# Autodesk Inventor assembly: CyberOrto
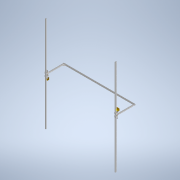
[picture p0: Inventor's stored thumbnail of the model, 180x180]
Saved by Autodesk Inventor 2022 (Build 260153000, 153)
## iProperties
RuleStatus: InUse
Created: 2021-12-29
Part Number: CyberOrto
Document SubType Name: Assembly
Designer: matte
Author: matte
## Documents named in this file (23)
- C:\Users\Elia\Documents\ELIA\UNITN\MAGISTRALE\1st year\1st semester\Mechanical Design\MDM-CyberOrto-CAD\CyberOrto.iam
- C:\Users\Elia\Documents\ELIA\UNITN\MAGISTRALE\1st year\1st semester\Mechanical Design\MDM-CyberOrto-CAD\Pezzi singoli\Trave Principale.ipt
- C:\Users\Elia\Documents\ELIA\UNITN\MAGISTRALE\1st year\1st semester\Mechanical Design\MDM-CyberOrto-CAD\Pezzi singoli\Supporto SX.ipt
- C:\Users\Elia\Documents\ELIA\UNITN\MAGISTRALE\1st year\1st semester\Mechanical Design\MDM-CyberOrto-CAD\Parker components\03-Brackets_Gussets_Plates\09-Machined Gussets\20-102.ipt
- C:\Users\Elia\Documents\ELIA\UNITN\MAGISTRALE\1st year\1st semester\Mechanical Design\MDM-CyberOrto-CAD\Parker components\02-Fasteners\10-Standard T-Nuts\20-050.ipt
- C:\Users\Elia\Documents\ELIA\UNITN\MAGISTRALE\1st year\1st semester\Mechanical Design\MDM-CyberOrto-CAD\Parker components\02-Fasteners\16-Screws\01-Metric Screws\01-Button Head\24-118-8.ipt
- C:\Users\Elia\Documents\ELIA\UNITN\MAGISTRALE\1st year\1st semester\Mechanical Design\MDM-CyberOrto-CAD\Guida a terra.iam
- C:\Users\Elia\Documents\ELIA\UNITN\MAGISTRALE\1st year\1st semester\Mechanical Design\MDM-CyberOrto-CAD\Parker components\05-Handles_Hinges\13-Pivot Joints\23-010.iam
- C:\Users\Elia\Documents\ELIA\UNITN\MAGISTRALE\1st year\1st semester\Mechanical Design\MDM-CyberOrto-CAD\Parker components\02-Fasteners\10-Standard T-Nuts\20-058.ipt
- C:\Users\Elia\Documents\ELIA\UNITN\MAGISTRALE\1st year\1st semester\Mechanical Design\MDM-CyberOrto-CAD\Parker components\02-Fasteners\16-Screws\01-Metric Screws\01-Button Head\24-116-8.ipt
- C:\Users\Elia\Documents\ELIA\UNITN\MAGISTRALE\1st year\1st semester\Mechanical Design\MDM-CyberOrto-CAD\Pezzi singoli\Supporto DX.ipt
- C:\Users\Elia\Documents\ELIA\UNITN\MAGISTRALE\1st year\1st semester\Mechanical Design\MDM-CyberOrto-CAD\Parker components\02-Fasteners\16-Screws\01-Metric Screws\01-Button Head\24-120-8.ipt
- C:\Users\Elia\Documents\ELIA\UNITN\MAGISTRALE\1st year\1st semester\Mechanical Design\MDM-CyberOrto-CAD\Pezzi singoli\Supporto lineare\Carrello semplice.iam
- C:\Users\Elia\Documents\ELIA\UNITN\MAGISTRALE\1st year\1st semester\Mechanical Design\MDM-CyberOrto-CAD\Platform.ipt
- C:\Users\Elia\Documents\ELIA\UNITN\MAGISTRALE\1st year\1st semester\Mechanical Design\MDM-CyberOrto-CAD\Parker components\02-Fasteners\16-Screws\01-Metric Screws\01-Button Head\24-130-6.ipt
- C:\Users\Elia\Documents\ELIA\UNITN\MAGISTRALE\1st year\1st semester\Mechanical Design\MDM-CyberOrto-CAD\Parker components\02-Fasteners\15-T-Bolts_Nuts_Washers\03-Washers\24-700-6.ipt
- C:\Users\Elia\Documents\ELIA\UNITN\MAGISTRALE\1st year\1st semester\Mechanical Design\MDM-CyberOrto-CAD\Parker components\02-Fasteners\15-T-Bolts_Nuts_Washers\02-Nuts\24-706-6.ipt
- C:\Users\Elia\Documents\ELIA\UNITN\MAGISTRALE\1st year\1st semester\Mechanical Design\MDM-CyberOrto-CAD\Servo Motor 50W\bch2mba531ca5c.ipt
- C:\Users\Elia\Documents\ELIA\UNITN\MAGISTRALE\1st year\1st semester\Mechanical Design\MDM-CyberOrto-CAD\Rack_Pinion\Rack gear scaled1.ipt
- C:\Users\Elia\Documents\ELIA\UNITN\MAGISTRALE\1st year\1st semester\Mechanical Design\MDM-CyberOrto-CAD\Rack_Pinion\pinion_scaled1.ipt
- C:\Users\Elia\Documents\ELIA\UNITN\MAGISTRALE\1st year\1st semester\Mechanical Design\MDM-CyberOrto-CAD\Inventor Support\Content Center Files\it-IT\ISO 1580\ISO 1580 - M4 x 12_.ipt
- C:\Users\Elia\Documents\ELIA\UNITN\MAGISTRALE\1st year\1st semester\Mechanical Design\MDM-CyberOrto-CAD\Inventor Support\Content Center Files\it-IT\AS 1474(1)\AS 1474 - M4(1).ipt
- C:\Users\Elia\Documents\ELIA\UNITN\MAGISTRALE\1st year\1st semester\Mechanical Design\MDM-CyberOrto-CAD\Trave a terra\Trave a terra.iam
## Components (89 placed, 22 different names)
1. Trave Principale:1 — Coincidente:1, Coincidente:2, Coincidente:3, Allineato:1, Coincidente:4, Allineato:2, Coincidente:5, Coincidente:10, Coincidente:40, Allineato:5, Allineato:6, Coincidente:41, Angolo:1
2. Supporto SX:1 — Allineato:1, Coincidente:4, Allineato:2, Coincidente:6, Allineato:3, Coincidente:7, Coincidente:15, Coincidente:16, Coincidente:23, Coincidente:28, Coincidente:29, Coincidente:30
3. Supporto DX:1 — Coincidente:45, Allineato:7, Allineato:8, Coincidente:48, Allineato:9, Allineato:10
4. Trave a terra:1 [sub-assembly] — Angolo:2, Angolo:3, Angolo:4, Allineato:59, Coincidente:130, Coincidente:131, Angolo:5, Allineato:60
5. 24-118-8:3 — Coincidente:19, Coincidente:20
6. 24-118-8:4 — Coincidente:21, Coincidente:22
7. 20-050:2 — Coincidente:10, Coincidente:11, Coincidente:12
8. 24-118-8:1 — Coincidente:13, Coincidente:14
9. 24-118-8:2 — Coincidente:17, Coincidente:18
10. 20-102:1 — Coincidente:5, Coincidente:6, Allineato:3, Coincidente:8, Coincidente:9, Coincidente:11, Coincidente:12, Coincidente:13, Coincidente:14, Coincidente:17, Coincidente:18, Coincidente:19, Coincidente:20, Coincidente:21, Coincidente:22
11. 20-050:1 — Coincidente:7, Coincidente:8, Coincidente:9
12. 24-118-8:5 — Coincidente:31, Coincidente:32, Coincidente:33
13. 24-118-8:6 — Coincidente:34, Coincidente:35
14. 24-118-8:7 — Coincidente:38, Coincidente:39
15. 24-118-8:8 — Coincidente:36, Coincidente:37
16. Guida a terra:1 [sub-assembly] — Coincidente:15, Coincidente:16, Coincidente:23, Coincidente:32, Coincidente:33, Coincidente:34, Coincidente:35, Coincidente:36, Coincidente:37, Coincidente:38, Coincidente:39, Coincidente:138, Coincidente:139, Allineato:61, Coincidente:141, Coincidente:143, Coincidente:145, Coincidente:162
17. 20-050:3 — Coincidente:27, Allineato:4, Coincidente:28, Coincidente:30, Coincidente:31
18. 20-050:4 — Coincidente:27, Allineato:4, Coincidente:29
19. 23-010:1 [sub-assembly] — Coincidente:40, Allineato:5, Allineato:6, Coincidente:43, Coincidente:44, Coincidente:45, Allineato:7, Allineato:8, Coincidente:46, Coincidente:47
20. 20-058:1 — Coincidente:41, Angolo:1, Coincidente:42
21. 24-116-8:1 — Coincidente:42, Coincidente:43, Coincidente:44
22. 24-120-8:1 — Coincidente:46, Coincidente:47
23. 24-120-8:2 — Coincidente:51, Coincidente:52
24. Carrello semplice:1 [sub-assembly] — Coincidente:48, Allineato:9, Allineato:10, Coincidente:51, Coincidente:52, Coincidente:53, Allineato:13, Coincidente:54, Coincidente:56, Coincidente:58, Coincidente:60, Coincidente:62, Angolo:2, Angolo:3, Angolo:4, Allineato:59, Coincidente:130
25. 24-130-6:1 — Inserimento:1, Coincidente:61
26. 24-700-6:1 — Inserimento:1, Inserimento:7
27. 24-706-6:1 — Coincidente:55, Coincidente:56
28. 24-130-6:2 — Coincidente:59
29. 24-700-6:3 — Inserimento:6
30. 24-130-6:3 — Coincidente:57
31. 24-700-6:2 — Inserimento:8
32. 24-130-6:4 — Coincidente:55
33. 24-700-6:4 — Inserimento:5
34. 24-706-6:2 — Coincidente:57, Coincidente:58
35. 24-706-6:3 — Coincidente:61, Coincidente:62
36. 24-706-6:4 — Coincidente:59, Coincidente:60
37. Platform:1 — Coincidente:53, Allineato:13, Coincidente:54, Inserimento:5, Inserimento:6, Inserimento:7, Inserimento:8, Coincidente:63, Coincidente:64, Coincidente:65, Coincidente:66, Coincidente:67, Coincidente:68, Coincidente:114, Coincidente:117, Coincidente:121, Coincidente:125, Coincidente:129
38. ISO 1580 M4 x 12:2 — Coincidente:126, Coincidente:127, Coincidente:128
39. AS 1474 - Metrico M4:2 — Coincidente:120, Coincidente:121
40. AS 1474 - Metrico M4:3 — Coincidente:124, Coincidente:125
41. AS 1474 - Metrico M4:4 — Coincidente:128, Coincidente:129
42. ISO 1580 M4 x 12:4 — Coincidente:118, Coincidente:119, Coincidente:120
43. ISO 1580 M4 x 12:3 — Coincidente:122, Coincidente:123, Coincidente:124
44. AS 1474 - Metrico M4:1 — Coincidente:116, Coincidente:117
45. ISO 1580 M4 x 12:1 — Coincidente:114, Coincidente:115, Coincidente:116
46. bch2mba531ca5c:1 — Coincidente:66, Coincidente:67, Coincidente:68, Coincidente:113, Coincidente:115, Coincidente:118, Coincidente:119, Coincidente:122, Coincidente:123, Coincidente:126, Coincidente:127
47. Rack gear scaled1:4 — Coincidente:74, Allineato:15, Coincidente:108, Allineato:33, Allineato:45, Allineato:46
48. Rack gear scaled1:5 — Coincidente:77, Allineato:17, Allineato:18, Coincidente:80, Allineato:42, Allineato:43, Angolo:5
49. Rack gear scaled1:6 — Coincidente:75, Allineato:16, Coincidente:77, Allineato:17, Allineato:43, Allineato:44
50. Rack gear scaled1:7 — Allineato:19, Coincidente:82, Allineato:20, Coincidente:83, Allineato:40, Allineato:41
51. Rack gear scaled1:8 — Coincidente:74, Allineato:15, Coincidente:75, Allineato:16, Allineato:44, Allineato:45
52. Rack gear scaled1:9 — Allineato:18, Coincidente:80, Allineato:19, Coincidente:82, Allineato:41, Allineato:42
53. Rack gear scaled1:10 — Coincidente:86, Allineato:21, Coincidente:89, Allineato:22, Allineato:38, Allineato:39
54. Rack gear scaled1:11 — Allineato:20, Coincidente:83, Coincidente:86, Allineato:21, Allineato:39, Allineato:40
55. Rack gear scaled1:12 — Coincidente:92, Allineato:24, Coincidente:94, Allineato:25, Allineato:47, Allineato:48, Allineato:49, Allineato:50, Allineato:51
56. Rack gear scaled1:13 — Coincidente:89, Allineato:22, Allineato:38, Allineato:60
57. Rack gear scaled1:14 — Coincidente:92, Allineato:24, Coincidente:108, Allineato:33, Allineato:36, Allineato:37, Allineato:46, Allineato:47
58. Rack gear scaled1:15 — Coincidente:94, Allineato:25, Coincidente:97, Allineato:26, Allineato:51
59. Rack gear scaled1:16 — Coincidente:97, Allineato:26, Coincidente:98, Allineato:27, Allineato:48, Allineato:49, Allineato:50, Allineato:52
60. Rack gear scaled1:17 — Coincidente:98, Allineato:27, Coincidente:101, Allineato:28, Allineato:52, Allineato:53
61. Rack gear scaled1:19 — Coincidente:105, Allineato:30, Coincidente:106, Allineato:31, Allineato:55, Allineato:56
62. Rack gear scaled1:20 — Coincidente:102, Allineato:29, Coincidente:105, Allineato:30, Allineato:54, Allineato:55
63. Rack gear scaled1:18 — Coincidente:101, Allineato:28, Coincidente:102, Allineato:29, Allineato:53, Allineato:54, Coincidente:131
64. Rack gear scaled1:21 — Coincidente:106, Allineato:31, Coincidente:109, Allineato:34, Allineato:56, Allineato:57
65. Rack gear scaled1:22 — Coincidente:109, Allineato:34, Coincidente:111, Allineato:35, Allineato:57, Allineato:58
66. Rack gear scaled1:23 — Coincidente:111, Allineato:35, Allineato:58
67. pinion_scaled1:1 — Coincidente:113, Allineato:36, Tangente:1
68. 24-706-6:8 — Coincidente:142, Coincidente:143
69. 24-706-6:7 — Coincidente:140, Coincidente:141
70. 24-706-6:6 — Coincidente:144, Coincidente:145
71. 24-700-6:8
72. 24-130-6:8 — Coincidente:146
73. 24-700-6:7
74. 24-130-6:7 — Coincidente:144
75. 24-700-6:6
76. 24-706-6:5 — Coincidente:146, Coincidente:162
77. 24-700-6:5
78. Platform:3 — Coincidente:138, Coincidente:139, Allineato:61, Coincidente:158, Coincidente:159, Coincidente:160, Coincidente:164
79. 24-130-6:5 — Coincidente:142
80. 24-130-6:6 — Coincidente:140
81. bch2mba531ca5c:2 — Coincidente:158, Coincidente:161
82. ISO 1580 M4 x 12:5 — Coincidente:161
83. AS 1474 - Metrico M4:5
84. ISO 1580 M4 x 12:6 — Coincidente:159, Coincidente:163
85. AS 1474 - Metrico M4:6
86. AS 1474 - Metrico M4:7
87. ISO 1580 M4 x 12:7
88. AS 1474 - Metrico M4:8 — Coincidente:163, Coincidente:164
89. ISO 1580 M4 x 12:8 — Coincidente:160
## Relationships (205: Mate 127, Flush 56, Insert 16, Angle 5, Tangent 1)
- Coincidente:1 [Mate]: Trave Principale:1
- Coincidente:2 [Mate]: Trave Principale:1
- Coincidente:3 [Mate]: Trave Principale:1
- Allineato:1 [Flush]: Trave Principale:1 ↔ Supporto SX:1
- Coincidente:4 [Mate]: Trave Principale:1 ↔ Supporto SX:1
- Allineato:2 [Flush]: Trave Principale:1 ↔ Supporto SX:1
- Coincidente:5 [Mate]: Trave Principale:1 ↔ 20-102:1
- Coincidente:6 [Mate]: Supporto SX:1 ↔ 20-102:1
- Allineato:3 [Flush]: Supporto SX:1 ↔ 20-102:1
- Coincidente:7 [Mate]: Supporto SX:1 ↔ 20-050:1
- Coincidente:8 [Mate]: 20-102:1 ↔ 20-050:1
- Coincidente:9 [Mate]: 20-102:1 ↔ 20-050:1
- Coincidente:10 [Mate]: Trave Principale:1 ↔ 20-050:2
- Coincidente:11 [Mate]: 20-050:2 ↔ 20-102:1
- Coincidente:12 [Mate]: 20-050:2 ↔ 20-102:1
- Coincidente:13 [Mate]: 24-118-8:1 ↔ 20-102:1
- Coincidente:14 [Mate]: 24-118-8:1 ↔ 20-102:1
- Coincidente:15 [Mate]: Supporto SX:1 ↔ Guida a terra:1
- Coincidente:16 [Mate]: Supporto SX:1 ↔ Guida a terra:1
- Coincidente:17 [Mate]: 24-118-8:2 ↔ 20-102:1
- Coincidente:18 [Mate]: 24-118-8:2 ↔ 20-102:1
- Coincidente:19 [Mate]: 24-118-8:3 ↔ 20-102:1
- Coincidente:20 [Mate]: 24-118-8:3 ↔ 20-102:1
- Coincidente:21 [Mate]: 24-118-8:4 ↔ 20-102:1
- Coincidente:22 [Mate]: 24-118-8:4 ↔ 20-102:1
- Coincidente:23 [Mate]: Supporto SX:1 ↔ Guida a terra:1
- Coincidente:27 [Mate]: 20-050:3 ↔ 20-050:4
- Allineato:4 [Flush]: 20-050:3 ↔ 20-050:4
- Coincidente:28 [Mate]: Supporto SX:1 ↔ 20-050:3
- Coincidente:29 [Mate]: Supporto SX:1 ↔ 20-050:4
- Coincidente:30 [Mate]: Supporto SX:1 ↔ 20-050:3
- Coincidente:31 [Mate]: 24-118-8:5 ↔ 20-050:3
- Coincidente:32 [Mate]: 24-118-8:5 ↔ Guida a terra:1
- Coincidente:33 [Mate]: 24-118-8:5 ↔ Guida a terra:1
- Coincidente:34 [Mate]: 24-118-8:6 ↔ Guida a terra:1
- Coincidente:35 [Mate]: 24-118-8:6 ↔ Guida a terra:1
- Coincidente:36 [Mate]: 24-118-8:8 ↔ Guida a terra:1
- Coincidente:37 [Mate]: 24-118-8:8 ↔ Guida a terra:1
- Coincidente:38 [Mate]: 24-118-8:7 ↔ Guida a terra:1
- Coincidente:39 [Mate]: 24-118-8:7 ↔ Guida a terra:1
- Coincidente:40 [Mate]: Trave Principale:1 ↔ 23-010:1
- Allineato:5 [Flush]: Trave Principale:1 ↔ 23-010:1
- Allineato:6 [Flush]: Trave Principale:1 ↔ 23-010:1
- Coincidente:41 [Mate]: Trave Principale:1 ↔ 20-058:1
- Angolo:1 [Angle] (0 deg): Trave Principale:1 ↔ 20-058:1
- Coincidente:42 [Mate]: 20-058:1 ↔ 24-116-8:1
- Coincidente:43 [Mate]: 23-010:1 ↔ 24-116-8:1
- Coincidente:44 [Mate]: 23-010:1 ↔ 24-116-8:1
- Coincidente:45 [Mate]: Supporto DX:1 ↔ 23-010:1
- Allineato:7 [Flush]: Supporto DX:1 ↔ 23-010:1
- Allineato:8 [Flush]: Supporto DX:1 ↔ 23-010:1
- Coincidente:46 [Mate]: 23-010:1 ↔ 24-120-8:1
- Coincidente:47 [Mate]: 23-010:1 ↔ 24-120-8:1
- Coincidente:48 [Mate]: Supporto DX:1 ↔ Carrello semplice:1
- Allineato:9 [Flush]: Supporto DX:1 ↔ Carrello semplice:1
- Allineato:10 [Flush]: Supporto DX:1 ↔ Carrello semplice:1
- Coincidente:51 [Mate]: 24-120-8:2 ↔ Carrello semplice:1
- Coincidente:52 [Mate]: 24-120-8:2 ↔ Carrello semplice:1
- Coincidente:53 [Mate]: Carrello semplice:1 ↔ Platform:1
- Allineato:13 [Flush]: Carrello semplice:1 ↔ Platform:1
- Coincidente:54 [Mate]: Carrello semplice:1 ↔ Platform:1
- Inserimento:1: 24-130-6:1 ↔ 24-700-6:1
- [Insert]: 24-130-6:2 ↔ 24-700-6:2
- [Insert]: 24-700-6:3 ↔ 24-130-6:3
- [Insert]: 24-130-6:4 ↔ 24-700-6:4
- Inserimento:5: 24-700-6:4 ↔ Platform:1
- Inserimento:6: 24-700-6:3 ↔ Platform:1
- Inserimento:7: 24-700-6:1 ↔ Platform:1
- Inserimento:8: 24-700-6:2 ↔ Platform:1
- Coincidente:55 [Mate]: 24-706-6:1 ↔ 24-130-6:4
- Coincidente:56 [Mate]: Carrello semplice:1 ↔ 24-706-6:1
- Coincidente:57 [Mate]: 24-130-6:3 ↔ 24-706-6:2
- Coincidente:58 [Mate]: Carrello semplice:1 ↔ 24-706-6:2
- Coincidente:59 [Mate]: 24-130-6:2 ↔ 24-706-6:4
- Coincidente:60 [Mate]: Carrello semplice:1 ↔ 24-706-6:4
- Coincidente:61 [Mate]: 24-130-6:1 ↔ 24-706-6:3
- Coincidente:62 [Mate]: Carrello semplice:1 ↔ 24-706-6:3
- Coincidente:63 [Mate]: Platform:1
- Coincidente:64 [Mate]: Platform:1
- Coincidente:65 [Mate]: Platform:1
- Coincidente:66 [Mate]: Platform:1 ↔ bch2mba531ca5c:1
- Coincidente:67 [Mate]: Platform:1 ↔ bch2mba531ca5c:1
- Coincidente:68 [Mate]: Platform:1 ↔ bch2mba531ca5c:1
- Coincidente:74 [Mate]: Rack gear scaled1:4 ↔ Rack gear scaled1:8
- Allineato:15 [Flush]: Rack gear scaled1:4 ↔ Rack gear scaled1:8
- Coincidente:75 [Mate]: Rack gear scaled1:6 ↔ Rack gear scaled1:8
- Allineato:16 [Flush]: Rack gear scaled1:6 ↔ Rack gear scaled1:8
- Coincidente:77 [Mate]: Rack gear scaled1:5 ↔ Rack gear scaled1:6
- Allineato:17 [Flush]: Rack gear scaled1:5 ↔ Rack gear scaled1:6
- Allineato:18 [Flush]: Rack gear scaled1:5 ↔ Rack gear scaled1:9
- Coincidente:80 [Mate]: Rack gear scaled1:5 ↔ Rack gear scaled1:9
- Allineato:19 [Flush]: Rack gear scaled1:7 ↔ Rack gear scaled1:9
- Coincidente:82 [Mate]: Rack gear scaled1:7 ↔ Rack gear scaled1:9
- Allineato:20 [Flush]: Rack gear scaled1:7 ↔ Rack gear scaled1:11
- Coincidente:83 [Mate]: Rack gear scaled1:7 ↔ Rack gear scaled1:11
- Coincidente:86 [Mate]: Rack gear scaled1:10 ↔ Rack gear scaled1:11
- Allineato:21 [Flush]: Rack gear scaled1:10 ↔ Rack gear scaled1:11
- Coincidente:89 [Mate]: Rack gear scaled1:10 ↔ Rack gear scaled1:13
- Allineato:22 [Flush]: Rack gear scaled1:10 ↔ Rack gear scaled1:13
- Coincidente:92 [Mate]: Rack gear scaled1:12 ↔ Rack gear scaled1:14
- Allineato:24 [Flush]: Rack gear scaled1:12 ↔ Rack gear scaled1:14
- Coincidente:94 [Mate]: Rack gear scaled1:12 ↔ Rack gear scaled1:15
- Allineato:25 [Flush]: Rack gear scaled1:12 ↔ Rack gear scaled1:15
- Coincidente:97 [Mate]: Rack gear scaled1:15 ↔ Rack gear scaled1:16
- Allineato:26 [Flush]: Rack gear scaled1:15 ↔ Rack gear scaled1:16
- Coincidente:98 [Mate]: Rack gear scaled1:16 ↔ Rack gear scaled1:17
- Allineato:27 [Flush]: Rack gear scaled1:16 ↔ Rack gear scaled1:17
- Coincidente:101 [Mate]: Rack gear scaled1:17 ↔ Rack gear scaled1:18
- Allineato:28 [Flush]: Rack gear scaled1:17 ↔ Rack gear scaled1:18
- Coincidente:102 [Mate]: Rack gear scaled1:20 ↔ Rack gear scaled1:18
- Allineato:29 [Flush]: Rack gear scaled1:20 ↔ Rack gear scaled1:18
- Coincidente:105 [Mate]: Rack gear scaled1:19 ↔ Rack gear scaled1:20
- Allineato:30 [Flush]: Rack gear scaled1:19 ↔ Rack gear scaled1:20
- Coincidente:106 [Mate]: Rack gear scaled1:19 ↔ Rack gear scaled1:21
- Allineato:31 [Flush]: Rack gear scaled1:19 ↔ Rack gear scaled1:21
- Coincidente:108 [Mate]: Rack gear scaled1:4 ↔ Rack gear scaled1:14
- Allineato:33 [Flush]: Rack gear scaled1:4 ↔ Rack gear scaled1:14
- Coincidente:109 [Mate]: Rack gear scaled1:21 ↔ Rack gear scaled1:22
- Allineato:34 [Flush]: Rack gear scaled1:21 ↔ Rack gear scaled1:22
- Coincidente:111 [Mate]: Rack gear scaled1:22 ↔ Rack gear scaled1:23
- Allineato:35 [Flush]: Rack gear scaled1:22 ↔ Rack gear scaled1:23
- Coincidente:113 [Mate]: bch2mba531ca5c:1 ↔ pinion_scaled1:1
- Allineato:36 [Flush]: Rack gear scaled1:14 ↔ pinion_scaled1:1
- Allineato:37 [Flush] (-0.9524 mm): Rack gear scaled1:14
- Tangente:1: pinion_scaled1:1
- Coincidente:114 [Mate]: Platform:1 ↔ ISO 1580 M4 x 12:1
- Coincidente:115 [Mate]: ISO 1580 M4 x 12:1 ↔ bch2mba531ca5c:1
- Coincidente:116 [Mate]: AS 1474 - Metrico M4:1 ↔ ISO 1580 M4 x 12:1
- Coincidente:117 [Mate]: Platform:1 ↔ AS 1474 - Metrico M4:1
- Coincidente:118 [Mate]: ISO 1580 M4 x 12:4 ↔ bch2mba531ca5c:1
- Coincidente:119 [Mate]: ISO 1580 M4 x 12:4 ↔ bch2mba531ca5c:1
- Coincidente:120 [Mate]: AS 1474 - Metrico M4:2 ↔ ISO 1580 M4 x 12:4
- Coincidente:121 [Mate]: Platform:1 ↔ AS 1474 - Metrico M4:2
- Coincidente:122 [Mate]: ISO 1580 M4 x 12:3 ↔ bch2mba531ca5c:1
- Coincidente:123 [Mate]: ISO 1580 M4 x 12:3 ↔ bch2mba531ca5c:1
- Coincidente:124 [Mate]: AS 1474 - Metrico M4:3 ↔ ISO 1580 M4 x 12:3
- Coincidente:125 [Mate]: Platform:1 ↔ AS 1474 - Metrico M4:3
- Coincidente:126 [Mate]: ISO 1580 M4 x 12:2 ↔ bch2mba531ca5c:1
- Coincidente:127 [Mate]: ISO 1580 M4 x 12:2 ↔ bch2mba531ca5c:1
- Coincidente:128 [Mate]: ISO 1580 M4 x 12:2 ↔ AS 1474 - Metrico M4:4
- Coincidente:129 [Mate]: Platform:1 ↔ AS 1474 - Metrico M4:4
- Allineato:38 [Flush]: Rack gear scaled1:10 ↔ Rack gear scaled1:13
- Allineato:39 [Flush]: Rack gear scaled1:10 ↔ Rack gear scaled1:11
- Allineato:40 [Flush]: Rack gear scaled1:7 ↔ Rack gear scaled1:11
- Allineato:41 [Flush]: Rack gear scaled1:7 ↔ Rack gear scaled1:9
- Allineato:42 [Flush]: Rack gear scaled1:5 ↔ Rack gear scaled1:9
- Allineato:43 [Flush]: Rack gear scaled1:5 ↔ Rack gear scaled1:6
- Allineato:44 [Flush]: Rack gear scaled1:6 ↔ Rack gear scaled1:8
- Allineato:45 [Flush]: Rack gear scaled1:4 ↔ Rack gear scaled1:8
- Allineato:46 [Flush]: Rack gear scaled1:4 ↔ Rack gear scaled1:14
- Allineato:47 [Flush]: Rack gear scaled1:12 ↔ Rack gear scaled1:14
- Allineato:48 [Flush]: Rack gear scaled1:12 ↔ Rack gear scaled1:16
- Allineato:49 [Flush]: Rack gear scaled1:12 ↔ Rack gear scaled1:16
- Allineato:50 [Flush]: Rack gear scaled1:12 ↔ Rack gear scaled1:16
- Allineato:51 [Flush]: Rack gear scaled1:12 ↔ Rack gear scaled1:15
- Allineato:52 [Flush]: Rack gear scaled1:16 ↔ Rack gear scaled1:17
- Allineato:53 [Flush]: Rack gear scaled1:17 ↔ Rack gear scaled1:18
- Allineato:54 [Flush]: Rack gear scaled1:20 ↔ Rack gear scaled1:18
- Allineato:55 [Flush]: Rack gear scaled1:19 ↔ Rack gear scaled1:20
- Allineato:56 [Flush]: Rack gear scaled1:19 ↔ Rack gear scaled1:21
- Allineato:57 [Flush]: Rack gear scaled1:21 ↔ Rack gear scaled1:22
- Allineato:58 [Flush]: Rack gear scaled1:22 ↔ Rack gear scaled1:23
- Angolo:2 [Angle] (0 deg): Trave a terra:1 ↔ Carrello semplice:1
- Angolo:3 [Angle] (0 deg): Trave a terra:1 ↔ Carrello semplice:1
- Angolo:4 [Angle] (0 deg): Trave a terra:1 ↔ Carrello semplice:1
- Allineato:59 [Flush] (19 mm): Trave a terra:1 ↔ Carrello semplice:1
- Coincidente:130 [Mate] (20 mm): Trave a terra:1 ↔ Carrello semplice:1
- Coincidente:131 [Mate]: Trave a terra:1 ↔ Rack gear scaled1:18
- Angolo:5 [Angle] (0 deg): Trave a terra:1 ↔ Rack gear scaled1:5
- Allineato:60 [Flush]: Trave a terra:1 ↔ Rack gear scaled1:13
- [Insert]: 24-700-6:5 ↔ 24-130-6:5
- [Insert]: 24-700-6:6 ↔ 24-130-6:6
- [Insert]: 24-700-6:7 ↔ 24-130-6:7
- [Insert]: 24-700-6:8 ↔ 24-130-6:8
- [Insert]: 24-700-6:8 ↔ Platform:3
- [Insert]: 24-700-6:7 ↔ Platform:3
- [Insert]: 24-700-6:5 ↔ Platform:3
- [Insert]: 24-700-6:6 ↔ Platform:3
- Coincidente:138 [Mate]: Guida a terra:1 ↔ Platform:3
- Coincidente:139 [Mate]: Guida a terra:1 ↔ Platform:3
- Allineato:61 [Flush]: Guida a terra:1 ↔ Platform:3
- Coincidente:140 [Mate]: 24-706-6:7 ↔ 24-130-6:6
- Coincidente:141 [Mate]: Guida a terra:1 ↔ 24-706-6:7
- Coincidente:142 [Mate]: 24-706-6:8 ↔ 24-130-6:5
- Coincidente:143 [Mate]: Guida a terra:1 ↔ 24-706-6:8
- Coincidente:144 [Mate]: 24-706-6:6 ↔ 24-130-6:7
- Coincidente:145 [Mate]: Guida a terra:1 ↔ 24-706-6:6
- Coincidente:146 [Mate]: 24-130-6:8 ↔ 24-706-6:5
- [Mate]: bch2mba531ca5c:2 ↔ ISO 1580 M4 x 12:5
- [Mate]: ISO 1580 M4 x 12:5 ↔ AS 1474 - Metrico M4:5
- [Mate]: bch2mba531ca5c:2 ↔ ISO 1580 M4 x 12:8
- [Mate]: bch2mba531ca5c:2 ↔ ISO 1580 M4 x 12:8
- [Mate]: AS 1474 - Metrico M4:6 ↔ ISO 1580 M4 x 12:8
- [Mate]: bch2mba531ca5c:2 ↔ ISO 1580 M4 x 12:7
- [Mate]: bch2mba531ca5c:2 ↔ ISO 1580 M4 x 12:7
- [Mate]: AS 1474 - Metrico M4:7 ↔ ISO 1580 M4 x 12:7
- [Mate]: bch2mba531ca5c:2 ↔ ISO 1580 M4 x 12:6
- [Mate]: bch2mba531ca5c:2 ↔ ISO 1580 M4 x 12:6
- Coincidente:158 [Mate]: Platform:3 ↔ bch2mba531ca5c:2
- Coincidente:159 [Mate]: Platform:3 ↔ ISO 1580 M4 x 12:6
- Coincidente:160 [Mate]: Platform:3 ↔ ISO 1580 M4 x 12:8
- Coincidente:161 [Mate]: bch2mba531ca5c:2 ↔ ISO 1580 M4 x 12:5
- Coincidente:162 [Mate]: Guida a terra:1 ↔ 24-706-6:5
- Coincidente:163 [Mate]: ISO 1580 M4 x 12:6 ↔ AS 1474 - Metrico M4:8
- Coincidente:164 [Mate]: Platform:3 ↔ AS 1474 - Metrico M4:8
## Named parameters: L_piatto_guide = 240 mm, L_tracce_terra = 4000 mm, L_traccia_superiore = 3000 mm, H_supporto = 700 mm, d116_d115 = 0 mm, d117_d115 = 0 mm, d118_d115 = 0 mm, d311_d115 = 0 mm, d312_d116_d115 = 0 mm, d313_d117_d115 = 0 mm, d314_d118_d115 = 0 mm, d315_d119 = 0 mm, d316_d120 = 0 mm, d317_d121 = 0 mm, d318_d122 = 0 mm, d333_d234 = 0 mm, d334_d235 = 0 mm, d335_d237 = 0 mm, d336_d238 = 0 mm, d337_d239 = 0 mm, d338_d241 = 0 mm, d339_d242 = 0 mm, d340_d243 = 0 mm, d341_d245 = 0 mm, d342_d246 = 0 mm
